# Autodesk Inventor assembly: Assembly2
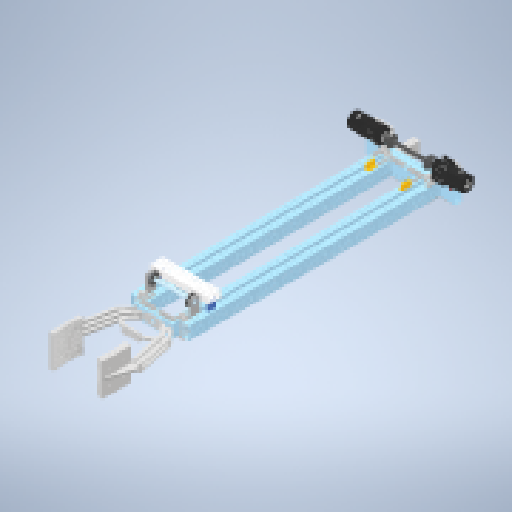
[picture p0: Inventor's stored thumbnail of the model, 512x512]
Saved by Autodesk Inventor 2023 (Build 270158000, 158)
## iProperties
Created: 2023-02-27
Part Number: Assembly2
Document SubType Name: Assembly
Designer: Gabriel - T3 CAD
Author: Gabriel - T3 CAD
## Documents named in this file (16)
- C:\Users\Gabriel - T3 CAD\Documents\GitHub\T3-CAD\New folder\Assembly2.iam
- C:\Users\Gabriel - T3 CAD\Documents\GitHub\T3-CAD\New folder\Pusher.ipt
- C:\Users\Gabriel - T3 CAD\Documents\GitHub\T3-CAD\New folder\Connector.ipt
- C:\Users\Gabriel - T3 CAD\Documents\GitHub\T3-CAD\New folder\Gripper triangle.ipt
- C:\Users\Gabriel - T3 CAD\Documents\GitHub\T3-CAD\New folder\Gripper plate.ipt
- C:\Users\Gabriel - T3 CAD\Documents\GitHub\T3-CAD\New folder\Pusher_MIR.ipt
- C:\Users\Gabriel - T3 CAD\Documents\GitHub\T3-CAD\New folder\Gripper triangle_MIR.ipt
- C:\Users\Gabriel - T3 CAD\Documents\GitHub\T3-CAD\New folder\Gripper plate_MIR.ipt
- C:\Users\Gabriel - T3 CAD\Documents\GitHub\T3-CAD\New folder\Face Plate.ipt
- C:\Users\Gabriel - T3 CAD\Documents\GitHub\T3-CAD\Current Season CAD\Swerve-DriveTrain-V2.1 (LongBot)\Potential new gripper\Gripper plate v2.ipt
- C:\Users\Gabriel - T3 CAD\Documents\GitHub\T3-CAD\Stock\ThriftyBot-Elevator\Configurable Thrifty Elevator_Simplify_2.ipt
- C:\Users\Gabriel - T3 CAD\Documents\GitHub\T3-CAD\Current Season CAD\Swerve-DriveTrain-V2.1 (LongBot)\Potential new gripper\Test  Stock Rotation extender.ipt
- C:\Users\Gabriel - T3 CAD\Documents\GitHub\T3-CAD\Stock\ThunderHex\Flanged Bearing.ipt
- C:\Users\Gabriel - T3 CAD\Documents\GitHub\T3-CAD\New folder\meth\standoff option1.ipt
- C:\Users\Gabriel - T3 CAD\Documents\GitHub\T3-CAD\New folder\meth\Part6.ipt
- C:\Users\Gabriel - T3 CAD\Documents\GitHub\T3-CAD\New folder\meth\PB OUT.ipt
## Components (21 placed, 15 different names)
1. Pusher:1 — Insert:3, Insert:51
2. Connector:1 — Insert:29, Insert:3, Insert:18, Insert:51, Insert:52
3. Gripper triangle:1 — Rigid:1
4. Gripper plate:1 — Rigid:1, Insert:26, Insert:28
5. Pusher_MIR:1 — Insert:18, Insert:52
6. Gripper triangle_MIR:1 — Rigid:2
7. Gripper plate_MIR:1 — Rigid:2, Insert:25, Insert:27
8. Face Plate:1 — Insert:29, Mate:13, Mate:14, Mate:15
9. Gripper plate v2:1 — Insert:26, Insert:28
10. Gripper plate v2:2 — Insert:25, Insert:27
11. Configurable Thrifty Elevator_Simplify_2:1 — Mate:3, Mate:4, Mate:5, Mate:6, Mate:7, Mate:8
12. Test  Stock Rotation extender:1 — Mate:1, Mate:2, Mate:3, Mate:4, Mate:5, Rotational:1, Rotational:4
13. Test  Stock Rotation extender:2 — Mate:1, Mate:2, Rotational:2, Rotational:3
14. Flanged Bearing:1 — Rotational:3
15. Flanged Bearing:2 — Rotational:2
16. Flanged Bearing:3 — Rotational:1
17. Flanged Bearing:4 — Rotational:4
18. standoff option1:1 — Mate:6, Mate:7, Mate:8, Mate:9, Mate:10, Mate:11, Mate:12
19. Part6:1 — Mate:9, Mate:12, Mate:13, Mate:14, Mate:15
20. Part6:2 — Mate:10, Mate:11
21. PB OUT:1
## Relationships (30: Mate 15, Insert 9, RevoluteJoint 4, WeldJoint 2)
- Insert:29 (19.8882 mm): Connector:1 ↔ Face Plate:1
- Insert:3: Pusher:1 ↔ Connector:1
- Rigid:1 [WeldJoint]: Gripper triangle:1 ↔ Gripper plate:1
- Rigid:2 [WeldJoint]: Gripper triangle_MIR:1 ↔ Gripper plate_MIR:1
- Insert:18: Connector:1 ↔ Pusher_MIR:1
- Insert:25: Gripper plate_MIR:1 ↔ Gripper plate v2:2
- Insert:26: Gripper plate:1 ↔ Gripper plate v2:1
- Insert:27: Gripper plate_MIR:1 ↔ Gripper plate v2:2
- Insert:28: Gripper plate:1 ↔ Gripper plate v2:1
- Mate:1 (127 mm): Test  Stock Rotation extender:1 ↔ Test  Stock Rotation extender:2
- Mate:2: Test  Stock Rotation extender:1 ↔ Test  Stock Rotation extender:2
- Mate:3: Configurable Thrifty Elevator_Simplify_2:1 ↔ Test  Stock Rotation extender:1
- Mate:4: Configurable Thrifty Elevator_Simplify_2:1 ↔ Test  Stock Rotation extender:1
- Mate:5 (88.9 mm): Configurable Thrifty Elevator_Simplify_2:1 ↔ Test  Stock Rotation extender:1
- Rotational:1 [RevoluteJoint]: Test  Stock Rotation extender:1 ↔ Flanged Bearing:3
- Rotational:2 [RevoluteJoint]: Test  Stock Rotation extender:2 ↔ Flanged Bearing:2
- Rotational:3 [RevoluteJoint]: Test  Stock Rotation extender:2 ↔ Flanged Bearing:1
- Rotational:4 [RevoluteJoint]: Test  Stock Rotation extender:1 ↔ Flanged Bearing:4
- Insert:51: Pusher:1 ↔ Connector:1
- Insert:52: Connector:1 ↔ Pusher_MIR:1
- Mate:6: Configurable Thrifty Elevator_Simplify_2:1 ↔ standoff option1:1
- Mate:7: Configurable Thrifty Elevator_Simplify_2:1 ↔ standoff option1:1
- Mate:8 (101.6 mm): Configurable Thrifty Elevator_Simplify_2:1 ↔ standoff option1:1
- Mate:9: standoff option1:1 ↔ Part6:1
- Mate:10: standoff option1:1 ↔ Part6:2
- Mate:11: standoff option1:1 ↔ Part6:2
- Mate:12: standoff option1:1 ↔ Part6:1
- Mate:13: Face Plate:1 ↔ Part6:1
- Mate:14: Face Plate:1 ↔ Part6:1
- Mate:15 (50.8 mm): Face Plate:1 ↔ Part6:1
